# Autodesk Inventor assembly: カウンター展開システム
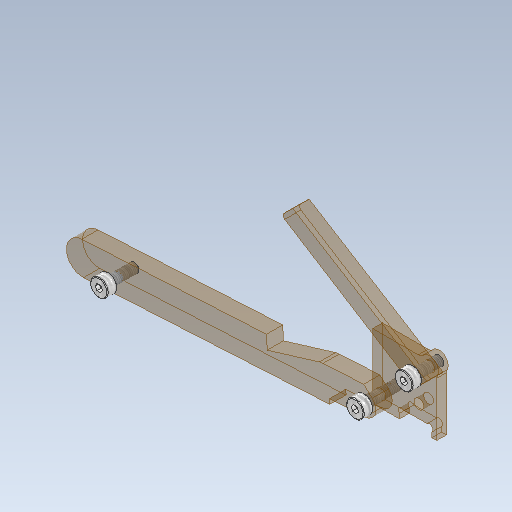
[picture p0: Inventor's stored thumbnail of the model, 512x512]
Saved by Autodesk Inventor 2020.2 (Build 242310000, 310)
## iProperties
Created: 2020-04-03
Part Number: カウンター展開システム
Document SubType Name: Assembly
Designer: aoyama
Mass: 8.99488 g
Surface Area: 55.3605 cm^2
Volume: 6.96361 cm^3
Density: 1.2917 g/cm^3
Author: aoyama
## Documents named in this file (6)
- C:\Users\aoyam\Desktop\SRDC_local\Inventor\二年機\インナー4層丙参型\全体\カウンター展開システム.iam
- C:\Users\aoyam\Desktop\SRDC_local\Inventor\二年機\インナー4層丙参型\全体\カウンター.ipt
- C:\Users\aoyam\Desktop\SRDC_local\Inventor\二年機\インナー4層丙参型\全体\カウンター展開.ipt
- C:\Users\aoyam\Desktop\SRDC_local\Inventor\二年機\インナー4層丙参型\全体\カウンター展開支柱test.ipt
- C:\Users\aoyam\Desktop\SRDC_local\Inventor\二年機\インナー4層丙参型\汎用部品\ネジアルミM3L8.ipt
- C:\Users\aoyam\Desktop\SRDC_local\Inventor\二年機\インナー4層丙参型\汎用部品\ネジアルミM3L12.ipt
## Components (6 placed, 5 different names)
1. カウンター:1 — 挿入:3, 挿入:14, 挿入:15
2. カウンター展開:1 — 挿入:11, 挿入:13
3. カウンター展開支柱test:1 — 挿入:3, 挿入:11
4. ネジアルミM3L8:2 — 挿入:13
5. ネジアルミM3L12:1 — 挿入:14
6. ネジアルミM3L8:3 — 挿入:15
## Relationships (5: Insert 5)
- 挿入:3 [Insert]: カウンター:1 ↔ カウンター展開支柱test:1
- 挿入:11 [Insert]: カウンター展開:1 ↔ カウンター展開支柱test:1
- 挿入:13 [Insert]: カウンター展開:1 ↔ ネジアルミM3L8:2
- 挿入:14 [Insert]: カウンター:1 ↔ ネジアルミM3L12:1
- 挿入:15 [Insert] (3 mm): カウンター:1 ↔ ネジアルミM3L8:3
